# Autodesk Inventor assembly: complete_assembly
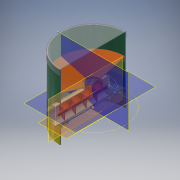
[picture p0: Inventor's stored thumbnail of the model, 180x180]
Saved by Autodesk Inventor 2019 (Build 230136000, 136)
## iProperties
Created: 2019-05-05
Part Number: complete_assembly
Document SubType Name: Assembly
Designer: assman
Author: assman
## Documents named in this file (9)
- D:\Inventor\Projects\CatFeeder\Case\version7\complete_assembly.iam
- D:\Inventor\Projects\CatFeeder\Case\version7\base.ipt
- D:\Inventor\Projects\CatFeeder\Case\version7\case.ipt
- D:\Inventor\Projects\CatFeeder\Case\version7\cap.ipt
- D:\Inventor\Projects\CatFeeder\Case\version7\inner_cone.ipt
- D:\Inventor\Projects\CatFeeder\Case\version7\auger_assembly.iam
- D:\Inventor\Projects\CatFeeder\Case\version6\esp8266_footprint.ipt
- D:\Inventor\Projects\CatFeeder\Case\version6\motordriver_footprint.ipt
- D:\Inventor\Projects\CatFeeder\Case\version7\cap_v2.ipt
## Components (8 placed, 8 different names)
1. base:1
2. case:1 — Rigid:1, Flush:1, Rigid:2, Rigid:3, Flush:2
3. cap:1
4. inner_cone:1 — Cylindrical:1
5. auger_assembly:1 [sub-assembly] — Rigid:1, Cylindrical:1, Flush:1
6. esp8266_footprint:1 — Rigid:3
7. motordriver_footprint:1 — Rigid:2
8. cap_v2:1 — Flush:2
## Relationships (6: WeldJoint 3, Flush 2, CylindricalJoint 1)
- Rigid:1 [WeldJoint]: case:1 ↔ auger_assembly:1
- Cylindrical:1: inner_cone:1 ↔ auger_assembly:1
- Flush:1: case:1 ↔ auger_assembly:1
- Rigid:2 [WeldJoint]: case:1 ↔ motordriver_footprint:1
- Rigid:3 [WeldJoint]: case:1 ↔ esp8266_footprint:1
- Flush:2: case:1 ↔ cap_v2:1
